# Autodesk Inventor assembly: EyasSay_Ensamblaje_rotacion_v3
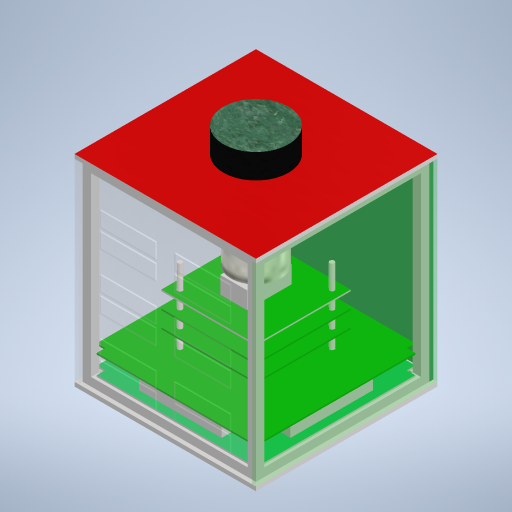
[picture p0: Inventor's stored thumbnail of the model, 512x512]
Saved by Autodesk Inventor 2024 (Build 280153000, 153)
## iProperties
Created: 2023-07-02
Part Number: EyasSay_Ensamblaje_rotacion_v3
Document SubType Name: Assembly
Designer: Personal
Author: Personal
## Documents named in this file (2)
- D:\Personal\Documents\GitHub\TDG_ReactionWheelsUnloading\Inventor\EyasSat_medicionesReales\EyasSay_Ensamblaje_rotacion_v3.iam
- D:\Personal\Documents\GitHub\TDG_ReactionWheelsUnloading\Inventor\EyasSat_medicionesReales\EyasSay_Ensamblaje_rotacion_v2.iam
## Components (1 placed, 1 different names)
1. EyasSay_Ensamblaje_rotacion_v2:1 [sub-assembly] — Coincidencia:1, Nivelación:1, Coincidencia:2
## Relationships (3: Mate 2, Flush 1)
- Coincidencia:1 [Mate]: EyasSay_Ensamblaje_rotacion_v2:1
- Nivelación:1 [Flush]: EyasSay_Ensamblaje_rotacion_v2:1
- Coincidencia:2 [Mate]: EyasSay_Ensamblaje_rotacion_v2:1
